# Autodesk Inventor assembly: PI-RACK-MOUNT
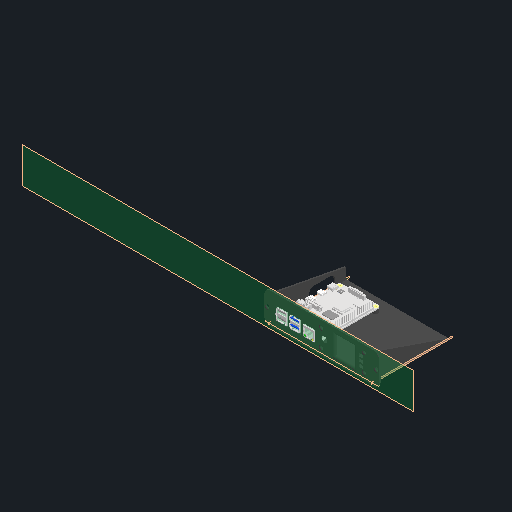
[picture p0: Inventor's stored thumbnail of the model, 512x512]
Saved by Autodesk Inventor 2026.2 (Build 302298010, 298A)
## iProperties
Created: 2026-03-25
Part Number: PI-RACK-MOUNT
Document SubType Name: Assembly
Designer: usr
Author: usr
## Documents named in this file (3)
- C:\Users\usr\Documents\IP-TERMINAL\PI-RACK-MOUNT.iam
- C:\Users\usr\Documents\IP-TERMINAL\Assembly2.iam
- C:\Users\usr\Documents\IP-TERMINAL\Raspberry Pi 4 Model B.iam
## Components (2 placed, 2 different names)
1. Assembly2:1 [sub-assembly] — Mate:1, Mate:2, Mate:3
2. Raspberry Pi 4 Model B:1 [sub-assembly] — Mate:1, Mate:2, Mate:3
## Relationships (3: Mate 3)
- Mate:1 (-3 mm): Assembly2:1 ↔ Raspberry Pi 4 Model B:1
- Mate:2 (5 mm): Assembly2:1 ↔ Raspberry Pi 4 Model B:1
- Mate:3 (5 mm): Assembly2:1 ↔ Raspberry Pi 4 Model B:1
